# Autodesk Inventor assembly: !battery_holder
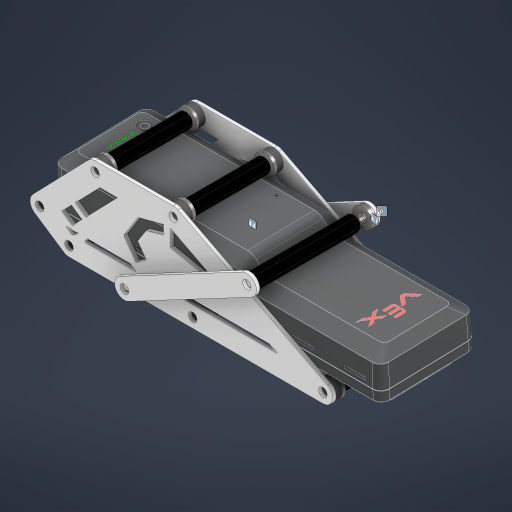
[picture p0: Inventor's stored thumbnail of the model, 512x512]
Saved by Autodesk Inventor 2024 (Build 280153000, 153)
## iProperties
Created: 2023-11-22
Part Number: !battery_holder
Document SubType Name: Assembly
Designer: avere
Author: avere
## Documents named in this file (12)
- C:\Users\avere\Documents\rbp_cad\zoomba_v0.1\chassis\!battery_holder.iam
- C:\Users\avere\Documents\rbp_cad\VEX-CAD-Inventor-1.41\Electronics\V5 Battery.ipt
- C:\Users\avere\Documents\rbp_cad\zoomba_v0.1\chassis\custom_parts\battery_mount_plate.ipt
- C:\Users\avere\Documents\rbp_cad\VEX-CAD-Inventor-1.41\Structure\Standoff\Standoff 1.50.ipt
- C:\Users\avere\Documents\rbp_cad\VEX-CAD-Inventor-1.41\Structure\Standoff.ipt
- C:\Users\avere\Documents\rbp_cad\VEX-CAD-Inventor-1.41\Motion\Spacers\Spacer Nylon .375 OD\NSpacer .375 OD x .125.ipt
- C:\Users\avere\Documents\rbp_cad\VEX-CAD-Inventor-1.41\Motion\Spacers\Spacer Nylon .375 OD.ipt
- C:\Users\avere\Documents\rbp_cad\VEX-CAD-Inventor-1.41\Motion\Spacers\Washer Steel\SWasher .375 OD x .062500.ipt
- C:\Users\avere\Documents\rbp_cad\VEX-CAD-Inventor-1.41\Motion\Spacers\Washer Steel.ipt
- C:\Users\avere\Documents\rbp_cad\zoomba_v0.1\chassis\custom_parts\battery_mount_arm.ipt
- C:\Users\avere\Documents\rbp_cad\VEX-CAD-Inventor-1.41\Structure\Standoff\Standoff 2.00.ipt
- C:\Users\avere\Documents\rbp_cad\VEX-CAD-Inventor-1.41\Motion\Spacers\Washer Steel\SWasher .375 OD x .031250.ipt
## Components (38 placed, 8 different names)
1. V5 Battery:1 — Mate:2
2. battery_mount_plate:1 — Insert:1, Insert:6, Mate:1, Insert:11, Insert:20, Insert:21, Insert:26, Mate:2, Insert:32
3. battery_mount_plate:2 — Insert:1, Mate:1, Insert:31, Insert:33
4. Standoff 1.50:1 — Insert:3, Insert:5
5. NSpacer .375 OD x .125:1 — Insert:2, Insert:6
6. SWasher .375 OD x .062500:1 — Insert:2, Insert:3
7. NSpacer .375 OD x .125:2
8. SWasher .375 OD x .062500:2 — Insert:5
9. Standoff 1.50:2
10. NSpacer .375 OD x .125:3 — Insert:11
11. SWasher .375 OD x .062500:3
12. NSpacer .375 OD x .125:4
13. SWasher .375 OD x .062500:4
14. Standoff 1.50:3
15. NSpacer .375 OD x .125:5 — Insert:21
16. SWasher .375 OD x .062500:5
17. NSpacer .375 OD x .125:6
18. SWasher .375 OD x .062500:6
19. Standoff 1.50:4
20. NSpacer .375 OD x .125:7 — Insert:20
21. SWasher .375 OD x .062500:7
22. NSpacer .375 OD x .125:8
23. SWasher .375 OD x .062500:8
24. Standoff 1.50:5
25. NSpacer .375 OD x .125:9 — Insert:26
26. SWasher .375 OD x .062500:9
27. NSpacer .375 OD x .125:10
28. SWasher .375 OD x .062500:10
29. Standoff 1.50:6
30. NSpacer .375 OD x .125:11 — Insert:31
31. SWasher .375 OD x .062500:11
32. NSpacer .375 OD x .125:12
33. SWasher .375 OD x .062500:12
34. battery_mount_arm:1 — Insert:32, Mate:3, Insert:37
35. battery_mount_arm:2 — Insert:33, Mate:3, Insert:38
36. Standoff 2.00:7 — Insert:37
37. SWasher .375 OD x .062500:13 — Insert:34
38. SWasher .375 OD x .031250:14 — Insert:34, Insert:38
## Relationships (39: Insert 36, Mate 3)
- Insert:1 (47.625 mm): battery_mount_plate:1 ↔ battery_mount_plate:2
- Insert:2: NSpacer .375 OD x .125:1 ↔ SWasher .375 OD x .062500:1
- Insert:3: Standoff 1.50:1 ↔ SWasher .375 OD x .062500:1
- [Insert]: NSpacer .375 OD x .125:2 ↔ SWasher .375 OD x .062500:2
- Insert:5: Standoff 1.50:1 ↔ SWasher .375 OD x .062500:2
- Insert:6: battery_mount_plate:1 ↔ NSpacer .375 OD x .125:1
- Mate:1: battery_mount_plate:1 ↔ battery_mount_plate:2
- [Insert]: NSpacer .375 OD x .125:3 ↔ SWasher .375 OD x .062500:3
- [Insert]: Standoff 1.50:2 ↔ SWasher .375 OD x .062500:3
- [Insert]: NSpacer .375 OD x .125:4 ↔ SWasher .375 OD x .062500:4
- [Insert]: Standoff 1.50:2 ↔ SWasher .375 OD x .062500:4
- Insert:11: battery_mount_plate:1 ↔ NSpacer .375 OD x .125:3
- [Insert]: NSpacer .375 OD x .125:5 ↔ SWasher .375 OD x .062500:5
- [Insert]: Standoff 1.50:3 ↔ SWasher .375 OD x .062500:5
- [Insert]: NSpacer .375 OD x .125:6 ↔ SWasher .375 OD x .062500:6
- [Insert]: Standoff 1.50:3 ↔ SWasher .375 OD x .062500:6
- [Insert]: NSpacer .375 OD x .125:7 ↔ SWasher .375 OD x .062500:7
- [Insert]: Standoff 1.50:4 ↔ SWasher .375 OD x .062500:7
- [Insert]: NSpacer .375 OD x .125:8 ↔ SWasher .375 OD x .062500:8
- [Insert]: Standoff 1.50:4 ↔ SWasher .375 OD x .062500:8
- Insert:20: battery_mount_plate:1 ↔ NSpacer .375 OD x .125:7
- Insert:21: battery_mount_plate:1 ↔ NSpacer .375 OD x .125:5
- [Insert]: NSpacer .375 OD x .125:9 ↔ SWasher .375 OD x .062500:9
- [Insert]: Standoff 1.50:5 ↔ SWasher .375 OD x .062500:9
- [Insert]: NSpacer .375 OD x .125:10 ↔ SWasher .375 OD x .062500:10
- [Insert]: Standoff 1.50:5 ↔ SWasher .375 OD x .062500:10
- Insert:26: battery_mount_plate:1 ↔ NSpacer .375 OD x .125:9
- Mate:2: V5 Battery:1 ↔ battery_mount_plate:1
- [Insert]: NSpacer .375 OD x .125:11 ↔ SWasher .375 OD x .062500:11
- [Insert]: Standoff 1.50:6 ↔ SWasher .375 OD x .062500:11
- [Insert]: NSpacer .375 OD x .125:12 ↔ SWasher .375 OD x .062500:12
- [Insert]: Standoff 1.50:6 ↔ SWasher .375 OD x .062500:12
- Insert:31: battery_mount_plate:2 ↔ NSpacer .375 OD x .125:11
- Insert:32 (3.175 mm): battery_mount_plate:1 ↔ battery_mount_arm:1
- Insert:33 (3.175 mm): battery_mount_plate:2 ↔ battery_mount_arm:2
- Mate:3: battery_mount_arm:1 ↔ battery_mount_arm:2
- Insert:34: SWasher .375 OD x .062500:13 ↔ SWasher .375 OD x .031250:14
- Insert:37: battery_mount_arm:1 ↔ Standoff 2.00:7
- Insert:38: battery_mount_arm:2 ↔ SWasher .375 OD x .031250:14
## Named parameters: d15_d13 = 0 mm, d19_d16 = 0 mm, d20_d13 = 0 mm, d21_d14 = 0 mm, d22_d15_d13 = 0 mm, d24_d16 = 0 mm, d25_d13 = 0 mm, d26_d14 = 0 mm, d27_d15_d13 = 0 mm, d28_d16 = 0 mm, d29_d13 = 0 mm, d30_d14 = 0 mm, d31_d15_d13 = 0 mm, d34_d24_d16 = 0 mm, d35_d25_d13 = 0 mm, d36_d26_d14 = 0 mm, d37_d27_d15_d13 = 0 mm, d40_d28_d16 = 0 mm, d41_d29_d13 = 0 mm, d42_d30_d14 = 0 mm, d43_d31_d15_d13 = 0 mm
